# Autodesk Inventor assembly: derived_drive_assembly_6_06_nn32
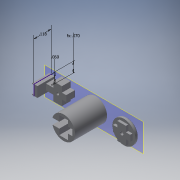
[picture p0: Inventor's stored thumbnail of the model, 180x180]
Saved by Autodesk Inventor 2016 (Build 200138000, 138)
## iProperties
Created: 2016-08-02
Part Number: derived_drive_assembly_6_06_nn32
Document SubType Name: Assembly
Designer: GentnerLab
Author: GentnerLab
## Documents named in this file (5)
- C:\Users\GentnerLab\Documents\Inventor\Parts\new_drive\60unm-6mm\derived_drive_assembly_6_06_nn32.iam
- C:\Users\GentnerLab\Documents\Inventor\Parts\new_drive\60unm-6mm\derived_body-6mm.ipt
- C:\Users\GentnerLab\Documents\Inventor\Parts\new_drive\60unm-6mm\derived_shuttle_6mm.ipt
- C:\Users\GentnerLab\Documents\Inventor\Parts\new_drive\60unm-6mm\derived_top_06mm.ipt
- C:\Users\GentnerLab\Documents\Inventor\Parts\new_drive\probe_carrier_nn32.ipt
## Components (4 placed, 4 different names)
1. derived_body-6mm:1 — Flush:1
2. derived_shuttle_6mm:1 — Flush:2, Mate:2, Mate:3, Mate:4
3. derived_top_06mm:1 — Mate:1
4. probe_carrier_nn32:1 — Mate:2, Mate:3, Mate:4
## Relationships (6: Mate 4, Flush 2)
- Flush:1: derived_body-6mm:1
- Mate:1: derived_top_06mm:1
- Flush:2: derived_shuttle_6mm:1
- Mate:2: derived_shuttle_6mm:1 ↔ probe_carrier_nn32:1
- Mate:3: derived_shuttle_6mm:1 ↔ probe_carrier_nn32:1
- Mate:4 (0.364 mm): derived_shuttle_6mm:1 ↔ probe_carrier_nn32:1
